# Autodesk Inventor assembly: full
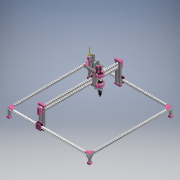
[picture p0: Inventor's stored thumbnail of the model, 180x180]
Saved by Autodesk Inventor 2019 (Build 230136000, 136)
## iProperties
Created: 2019-05-07
Part Number: full
Document SubType Name: Assembly
Designer: Alex Jones
Author: Alex Jones
## Documents named in this file (24)
- C:\Users\Alex Jones\Documents\Inventor\CNC\full.iam
- C:\Users\Alex Jones\Documents\Inventor\CNC\base.iam
- C:\Users\Alex Jones\Documents\Inventor\CNC\carriage.iam
- C:\Users\Alex Jones\Documents\Inventor\CNC\2020-1m.ipt
- C:\Users\Alex Jones\Documents\Inventor\CNC\cap.ipt
- C:\Users\Alex Jones\Documents\Inventor\CNC\2020-25cm.ipt
- C:\Users\Alex Jones\Documents\Inventor\CNC\double90.ipt
- C:\Users\Alex Jones\Documents\Inventor\CNC\bearingStandin.ipt
- C:\Users\Alex Jones\Documents\Inventor\CNC\couplerStandin.ipt
- C:\Users\Alex Jones\Documents\Inventor\CNC\nema17.ipt
- C:\Users\Alex Jones\Documents\Inventor\CNC\standinNut.ipt
- C:\Users\Alex Jones\Documents\Inventor\CNC\bed.iam
- C:\Users\Alex Jones\Documents\Inventor\CNC\roller.ipt
- C:\Users\Alex Jones\Documents\Inventor\CNC\yCarraige.ipt
- C:\Users\Alex Jones\Documents\Inventor\CNC\ZHolder.ipt
- C:\Users\Alex Jones\Documents\Inventor\CNC\threadedRodStandinShort.ipt
- C:\Users\Alex Jones\Documents\Inventor\CNC\Part3.ipt
- C:\Users\Alex Jones\Documents\Inventor\CNC\rollerHolderInnerZ.ipt
- C:\Users\Alex Jones\Documents\Inventor\CNC\Dremel.ipt
- C:\Users\Alex Jones\Documents\Inventor\CNC\DremelHolder.ipt
- C:\Users\Alex Jones\Documents\Inventor\CNC\dremelClamp.ipt
- C:\Users\Alex Jones\Documents\Inventor\CNC\ZNutHolder.ipt
- C:\Users\Alex Jones\Documents\Inventor\CNC\2020-125mm.ipt
- C:\Users\Alex Jones\Documents\Inventor\CNC\limitHolder.ipt
## Components (60 placed, 23 different names)
1. base:1 [sub-assembly] — Tangent:1, Tangent:2, Tangent:3, Tangent:4, Tangent:5, Tangent:6, Flush:19, Flush:40
2. carriage:1 [sub-assembly] — Tangent:5, Tangent:6, Flush:1, Mate:6, Mate:7, Mate:8
3. 2020-25cm:2 — Flush:8, Mate:8, Flush:9, Mate:22, Mate:40
4. 2020-25cm:1 — Mate:6, Flush:8, Mate:7, Mate:9, Mate:10, Mate:11, Flush:11, Mate:15, Mate:16, Mate:17, Mate:39
5. cap:1 — Flush:9, Mate:9, Mate:10, Mate:11
6. cap:2 — Mate:12, Mate:13, Mate:14
7. cap:3 — Mate:15, Mate:16, Mate:17
8. cap:4 — Mate:18, Mate:19, Mate:20, Mate:21
9. 2020-1m:5 — Mate:23, Flush:12, Flush:13, Mate:27, Mate:28, Mate:31, Mate:33, Flush:19, Flush:20, Flush:22, Tangent:11, Tangent:12, Tangent:13, Tangent:14, Angle:7, Mate:93, Mate:94, Angle:11
10. 2020-1m:6 — Mate:22, Mate:23, Flush:12, Flush:13, Mate:29, Mate:32, Mate:35, Tangent:15, Tangent:16, Tangent:17, Tangent:18, Mate:92
11. cap:6 — Mate:27, Mate:28, Mate:29
12. double90:1 — Mate:32, Mate:37, Flush:20, Flush:21
13. double90:2 — Mate:31, Mate:38, Flush:21
14. double90:3 — Mate:33, Mate:40, Flush:23
15. double90:4 — Mate:35, Mate:39, Flush:22, Flush:23
16. bed:1 [sub-assembly] — Flush:40
17. roller:1 — Tangent:17, Tangent:18, Mate:76, Mate:81, Mate:83
18. roller:2 — Tangent:15, Tangent:16, Mate:79
19. roller:3 — Tangent:13, Tangent:14, Mate:78, Mate:80, Mate:82, Mate:84, Mate:85
20. roller:4 — Tangent:11, Tangent:12, Mate:77
21. yCarraige:1 — Mate:80, Mate:81, Mate:85, Mate:86, Flush:43, Mate:87, Mate:88, Flush:44, Mate:89, Mate:114
22. yCarraige:2 — Mate:82, Mate:83, Mate:84, Mate:90, Flush:46, Flush:47, Mate:91, Flush:51
23. 2020-25cm:5 — Mate:88, Flush:44, Mate:89, Tangent:19, Tangent:20, Tangent:23, Tangent:24, Tangent:26, Tangent:27, Tangent:28, Tangent:29
24. 2020-25cm:6 — Mate:86, Flush:43, Mate:87, Tangent:21, Tangent:22, Tangent:25, Tangent:30, Tangent:31, Tangent:32, Tangent:33, Mate:115
25. 2020-25cm:7 — Mate:90, Flush:46, Mate:95, Mate:96, Mate:97, Mate:98, Flush:48, Flush:50, Mate:143, Flush:69, Flush:71
26. 2020-25cm:8 — Flush:47, Mate:91, Angle:8, Angle:9, Angle:10, Flush:48, Flush:53, Angle:15, Mate:142, Mate:144, Flush:70
27. cap:7 — Mate:92, Mate:93, Mate:94
28. bearingStandin:5 — Mate:95, Angle:8, Mate:96, Mate:99, Mate:100
29. bearingStandin:6 — Angle:9, Mate:97, Mate:98, Mate:102, Flush:53
30. nema17:3 — Mate:101, Angle:10, Flush:49, Mate:103, Flush:51, Mate:141
31. couplerStandin:3 — Mate:99, Mate:100, Mate:101, Flush:52
32. ZHolder:1 — Flush:49, Flush:50, Mate:141, Mate:142
33. threadedRodStandinShort:1 — Mate:102, Mate:103, Flush:52, Mate:104, Angle:12
34. standinNut:3 — Mate:104, Mate:136, Mate:137, Mate:140
35. roller:5 — Tangent:19, Tangent:20, Mate:105
36. roller:6 — Tangent:23, Tangent:24, Mate:106, Mate:121
37. roller:7 — Mate:106, Tangent:25, Mate:111
38. roller:8 — Tangent:21, Tangent:22, Mate:105, Mate:109, Mate:118
39. roller:9 — Tangent:26, Tangent:27, Mate:108, Mate:120
40. roller:10 — Tangent:28, Tangent:29, Mate:107, Mate:119
41. roller:11 — Tangent:30, Tangent:31, Mate:108, Mate:112, Mate:116, Mate:117
42. roller:12 — Tangent:32, Tangent:33, Mate:107, Mate:110
43. 2020-25cm:9 — Mate:114, Mate:115, Mate:122, Flush:55, Mate:124, Mate:125, Flush:56, Tangent:34, Mate:126, Mate:128, Flush:60, Mate:131, Flush:63
44. Part3:1 — Mate:116, Mate:117, Mate:118, Mate:123, Flush:66, Flush:67, Mate:135
45. Part3:2 — Mate:119, Mate:120, Mate:121, Flush:64, Mate:134, Flush:65
46. rollerHolderInnerZ:1 — Mate:122, Mate:123, Flush:55, Mate:124, Flush:57, Mate:127, Mate:132
47. rollerHolderInnerZ:2 — Mate:125, Flush:56, Flush:57
48. Dremel:1 — Tangent:34, Angle:12, Mate:126, Mate:127
49. DremelHolder:1 — Flush:59, Mate:128, Flush:60, Flush:61, Mate:129, Angle:13
50. dremelClamp:1 — Flush:61, Mate:129, Angle:13, Mate:132, Mate:133
51. DremelHolder:2 — Mate:131, Flush:63, Mate:133
52. dremelClamp:2
53. 2020-125mm:1 — Flush:64, Mate:134, Flush:65, Flush:68
54. 2020-125mm:2 — Flush:66, Flush:67, Mate:135
55. ZNutHolder:1 — Flush:68, Mate:140
56. limitHolder:1 — Mate:143, Flush:69, Flush:71
57. limitHolder:2 — Mate:144, Flush:70
58. 2020-25cm:3 — Mate:2, Mate:5, Flush:5, Flush:10, Flush:11, Mate:38
59. 2020-25cm:4 — Mate:4, Flush:5, Mate:12, Mate:13, Mate:14, Flush:10, Mate:18, Mate:19, Mate:20, Mate:37
60. carriage:2 [sub-assembly] — Tangent:1, Tangent:2, Tangent:3, Tangent:4, Flush:1, Mate:2, Mate:4, Mate:5, Mate:21
## Relationships (182: Mate 101, Flush 41, Tangent 30, Angle 10)
- Tangent:1: base:1 ↔ carriage:2
- Tangent:2: base:1 ↔ carriage:2
- Tangent:3: base:1 ↔ carriage:2
- Tangent:4: base:1 ↔ carriage:2
- Tangent:5: base:1 ↔ carriage:1
- Tangent:6: base:1 ↔ carriage:1
- Flush:1: carriage:1 ↔ carriage:2
- Mate:2 (-10 mm): 2020-25cm:3 ↔ carriage:2
- Mate:4 (-10 mm): 2020-25cm:4 ↔ carriage:2
- Mate:5: 2020-25cm:3 ↔ carriage:2
- Flush:5: 2020-25cm:3 ↔ 2020-25cm:4
- Mate:6: carriage:1 ↔ 2020-25cm:1
- Flush:8: 2020-25cm:2 ↔ 2020-25cm:1
- Mate:7 (-10 mm): carriage:1 ↔ 2020-25cm:1
- Mate:8 (-10 mm): carriage:1 ↔ 2020-25cm:2
- Flush:9: 2020-25cm:2 ↔ cap:1
- Mate:9: 2020-25cm:1 ↔ cap:1
- Mate:10: 2020-25cm:1 ↔ cap:1
- Mate:11: 2020-25cm:1 ↔ cap:1
- Mate:12: cap:2 ↔ 2020-25cm:4
- Mate:13: cap:2 ↔ 2020-25cm:4
- Mate:14: cap:2 ↔ 2020-25cm:4
- Flush:10: 2020-25cm:3 ↔ 2020-25cm:4
- Flush:11: 2020-25cm:1 ↔ 2020-25cm:3
- Mate:15: 2020-25cm:1 ↔ cap:3
- Mate:16: 2020-25cm:1 ↔ cap:3
- Mate:17: 2020-25cm:1 ↔ cap:3
- Mate:18: cap:4 ↔ 2020-25cm:4
- Mate:19: cap:4 ↔ 2020-25cm:4
- Mate:20: cap:4 ↔ 2020-25cm:4
- Mate:21 (1.27 mm): cap:4 ↔ carriage:2
- Mate:22: 2020-25cm:2 ↔ 2020-1m:6
- Mate:23 (20 mm): 2020-1m:5 ↔ 2020-1m:6
- Flush:12: 2020-1m:5 ↔ 2020-1m:6
- Flush:13: 2020-1m:5 ↔ 2020-1m:6
- Mate:27: 2020-1m:5 ↔ cap:6
- Mate:28: 2020-1m:5 ↔ cap:6
- Mate:29: 2020-1m:6 ↔ cap:6
- Mate:31: 2020-1m:5 ↔ double90:2
- Mate:32: 2020-1m:6 ↔ double90:1
- Mate:33: 2020-1m:5 ↔ double90:3
- Mate:35: 2020-1m:6 ↔ double90:4
- Flush:19: base:1 ↔ 2020-1m:5
- Mate:37: double90:1 ↔ 2020-25cm:4
- Flush:20: 2020-1m:5 ↔ double90:1
- Mate:38: double90:2 ↔ 2020-25cm:3
- Flush:21: double90:1 ↔ double90:2
- Mate:39: 2020-25cm:1 ↔ double90:4
- Flush:22: 2020-1m:5 ↔ double90:4
- Mate:40: 2020-25cm:2 ↔ double90:3
- Flush:23: double90:3 ↔ double90:4
- Flush:40: base:1 ↔ bed:1
- Tangent:11: 2020-1m:5 ↔ roller:4
- Tangent:12: 2020-1m:5 ↔ roller:4
- Tangent:13: 2020-1m:5 ↔ roller:3
- Tangent:14: 2020-1m:5 ↔ roller:3
- Tangent:15: 2020-1m:6 ↔ roller:2
- Tangent:16: 2020-1m:6 ↔ roller:2
- Tangent:17: 2020-1m:6 ↔ roller:1
- Tangent:18: 2020-1m:6 ↔ roller:1
- Mate:76: roller:1
- Mate:77: roller:4
- Mate:78: roller:3
- Mate:79: roller:2
- Angle:6 (0 deg)
- Angle:7 (90 deg): 2020-1m:5
- Flush:42 (-42 mm)
- Mate:80: roller:3 ↔ yCarraige:1
- Mate:81: roller:1 ↔ yCarraige:1
- Mate:82: roller:3 ↔ yCarraige:2
- Mate:83: roller:1 ↔ yCarraige:2
- Mate:84 (6 mm): roller:3 ↔ yCarraige:2
- Mate:85 (6 mm): roller:3 ↔ yCarraige:1
- Mate:86: yCarraige:1 ↔ 2020-25cm:6
- Flush:43: yCarraige:1 ↔ 2020-25cm:6
- Mate:87 (-10 mm): yCarraige:1 ↔ 2020-25cm:6
- Mate:88: yCarraige:1 ↔ 2020-25cm:5
- Flush:44: yCarraige:1 ↔ 2020-25cm:5
- Mate:89 (-10 mm): yCarraige:1 ↔ 2020-25cm:5
- Mate:90: yCarraige:2 ↔ 2020-25cm:7
- Flush:46: yCarraige:2 ↔ 2020-25cm:7
- Flush:47: yCarraige:2 ↔ 2020-25cm:8
- Mate:91: yCarraige:2 ↔ 2020-25cm:8
- Mate:92: 2020-1m:6 ↔ cap:7
- Mate:93: 2020-1m:5 ↔ cap:7
- Mate:94: 2020-1m:5 ↔ cap:7
- Mate:95: 2020-25cm:7 ↔ bearingStandin:5
- Angle:8 (0 deg): 2020-25cm:8 ↔ bearingStandin:5
- Mate:96 (-10 mm): 2020-25cm:7 ↔ bearingStandin:5
- Angle:9 (0 deg): 2020-25cm:8 ↔ bearingStandin:6
- Mate:97: 2020-25cm:7 ↔ bearingStandin:6
- Mate:98 (-10 mm): 2020-25cm:7 ↔ bearingStandin:6
- Mate:99: bearingStandin:5 ↔ couplerStandin:3
- Mate:100: bearingStandin:5 ↔ couplerStandin:3
- Mate:101: nema17:3 ↔ couplerStandin:3
- Angle:10 (45 deg): 2020-25cm:8 ↔ nema17:3
- Flush:48: 2020-25cm:7 ↔ 2020-25cm:8
- Flush:49: nema17:3 ↔ ZHolder:1
- Flush:50: 2020-25cm:7 ↔ ZHolder:1
- Mate:102: bearingStandin:6 ↔ threadedRodStandinShort:1
- Mate:103: nema17:3 ↔ threadedRodStandinShort:1
- Flush:51: yCarraige:2 ↔ nema17:3
- Flush:52 (-12 mm): couplerStandin:3 ↔ threadedRodStandinShort:1
- Flush:53 (15 mm): 2020-25cm:8 ↔ bearingStandin:6
- Mate:104: threadedRodStandinShort:1 ↔ standinNut:3
- Tangent:19: 2020-25cm:5 ↔ roller:5
- Tangent:20: 2020-25cm:5 ↔ roller:5
- Tangent:21: 2020-25cm:6 ↔ roller:8
- Tangent:22: 2020-25cm:6 ↔ roller:8
- Mate:105: roller:5 ↔ roller:8
- Tangent:23: 2020-25cm:5 ↔ roller:6
- Tangent:24: 2020-25cm:5 ↔ roller:6
- Mate:106: roller:6 ↔ roller:7
- Tangent:25: 2020-25cm:6 ↔ roller:7
- Tangent:26: 2020-25cm:5 ↔ roller:9
- Tangent:27: 2020-25cm:5 ↔ roller:9
- Tangent:28: 2020-25cm:5 ↔ roller:10
- Tangent:29: 2020-25cm:5 ↔ roller:10
- Tangent:30: 2020-25cm:6 ↔ roller:11
- Tangent:31: 2020-25cm:6 ↔ roller:11
- Tangent:32: 2020-25cm:6 ↔ roller:12
- Tangent:33: 2020-25cm:6 ↔ roller:12
- Mate:107: roller:10 ↔ roller:12
- Mate:108: roller:9 ↔ roller:11
- Mate:109: roller:8
- Mate:110: roller:12
- Mate:111: roller:7
- Mate:112: roller:11
- Angle:11 (0 deg): 2020-1m:5
- Mate:113 (25 mm)
- Mate:114: yCarraige:1 ↔ 2020-25cm:9
- Mate:115 (1 mm): 2020-25cm:6 ↔ 2020-25cm:9
- Mate:116 (6 mm): roller:11 ↔ Part3:1
- Mate:117: roller:11 ↔ Part3:1
- Mate:118: roller:8 ↔ Part3:1
- Mate:119: roller:10 ↔ Part3:2
- Mate:120 (6 mm): roller:9 ↔ Part3:2
- Mate:121: roller:6 ↔ Part3:2
- Mate:122: 2020-25cm:9 ↔ rollerHolderInnerZ:1
- Mate:123: Part3:1 ↔ rollerHolderInnerZ:1
- Flush:55: 2020-25cm:9 ↔ rollerHolderInnerZ:1
- Mate:124 (-10 mm): 2020-25cm:9 ↔ rollerHolderInnerZ:1
- Mate:125: 2020-25cm:9 ↔ rollerHolderInnerZ:2
- Flush:56: 2020-25cm:9 ↔ rollerHolderInnerZ:2
- Flush:57: rollerHolderInnerZ:1 ↔ rollerHolderInnerZ:2
- Tangent:34 (12.7 mm): 2020-25cm:9 ↔ Dremel:1
- Angle:12 (180 deg): threadedRodStandinShort:1 ↔ Dremel:1
- Mate:126 (-10 mm): 2020-25cm:9 ↔ Dremel:1
- Mate:127: rollerHolderInnerZ:1 ↔ Dremel:1
- Flush:59: DremelHolder:1
- Mate:128: 2020-25cm:9 ↔ DremelHolder:1
- Flush:60: 2020-25cm:9 ↔ DremelHolder:1
- Flush:61: DremelHolder:1 ↔ dremelClamp:1
- Mate:129: DremelHolder:1 ↔ dremelClamp:1
- Angle:13 (180 deg): DremelHolder:1 ↔ dremelClamp:1
- [Flush]: DremelHolder:2 ↔ dremelClamp:2
- [Mate]: DremelHolder:2 ↔ dremelClamp:2
- [Angle] (180 deg): DremelHolder:2 ↔ dremelClamp:2
- Mate:131: 2020-25cm:9 ↔ DremelHolder:2
- Flush:63: 2020-25cm:9 ↔ DremelHolder:2
- Mate:132: rollerHolderInnerZ:1 ↔ dremelClamp:1
- Mate:133 (76.2 mm): dremelClamp:1 ↔ DremelHolder:2
- Flush:64: Part3:2 ↔ 2020-125mm:1
- Mate:134: Part3:2 ↔ 2020-125mm:1
- Flush:65: Part3:2 ↔ 2020-125mm:1
- Flush:66: Part3:1 ↔ 2020-125mm:2
- Flush:67: Part3:1 ↔ 2020-125mm:2
- Mate:135: Part3:1 ↔ 2020-125mm:2
- Flush:68: 2020-125mm:1 ↔ ZNutHolder:1
- Mate:136: standinNut:3
- Mate:137: standinNut:3
- Mate:138
- Mate:139
- Angle:15 (0 deg): 2020-25cm:8
- Mate:140: standinNut:3 ↔ ZNutHolder:1
- Mate:141: nema17:3 ↔ ZHolder:1
- Mate:142: 2020-25cm:8 ↔ ZHolder:1
- Mate:143: 2020-25cm:7 ↔ limitHolder:1
- Flush:69: 2020-25cm:7 ↔ limitHolder:1
- Mate:144: 2020-25cm:8 ↔ limitHolder:2
- Flush:70: 2020-25cm:8 ↔ limitHolder:2
- Flush:71: 2020-25cm:7 ↔ limitHolder:1
## Named parameters: d327_d324 = 0 mm, d328_d325 = 0 mm, d329_d326 = 180 deg
